# Autodesk Inventor assembly: Tracker
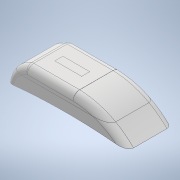
[picture p0: Inventor's stored thumbnail of the model, 180x180]
Saved by Autodesk Inventor 2020 (Build 240168000, 168)
## iProperties
Created: 2019-07-11
Part Number: Tracker
Document SubType Name: Assembly
Designer: tyrre
Author: tyrre
## Documents named in this file (6)
- C:\Users\tyrre\OneDrive\Desktop\University - Ryan\Work\Work - 2019\Inventor Files\Tracker V2\Tracker V2.iam
- C:\Users\tyrre\OneDrive\Desktop\University - Ryan\Work\Work - 2019\Inventor Files\Tracker V2\BatteryV2.ipt
- C:\Users\tyrre\OneDrive\Desktop\University - Ryan\Work\Work - 2019\Inventor Files\Tracker V2\GPSV2.ipt
- C:\Users\tyrre\OneDrive\Desktop\University - Ryan\Work\Work - 2019\Inventor Files\Tracker V2\MoteinoPCBV2.ipt
- C:\Users\tyrre\OneDrive\Desktop\University - Ryan\Work\Work - 2019\Inventor Files\Tracker V2\Case - BottomV2.ipt
- C:\Users\tyrre\OneDrive\Desktop\University - Ryan\Work\Work - 2019\Inventor Files\Tracker V2\Case - TopV2.ipt
## Components (5 placed, 5 different names)
1. Battery:1 — Mate:1, Flush:2, Flush:3, Flush:5, Mate:8, Mate:9
2. GPS:1 — Mate:2, Flush:4, Flush:5, Mate:6, Mate:7, Flush:6
3. MoteinoPCBV2:1 — Mate:1, Flush:2, Flush:3, Mate:2, Flush:4
4. Case - Top:1 — Mate:6, Mate:7, Mate:10, Flush:6
5. Case - Bottom:1 — Mate:8, Mate:9, Mate:10
## Relationships (12: Mate 7, Flush 5)
- Mate:1: Battery:1 ↔ MoteinoPCBV2:1
- Flush:2 (1.193 mm): Battery:1 ↔ MoteinoPCBV2:1
- Flush:3: Battery:1 ↔ MoteinoPCBV2:1
- Mate:2: GPS:1 ↔ MoteinoPCBV2:1
- Flush:4: GPS:1 ↔ MoteinoPCBV2:1
- Flush:5 (8.75 mm): Battery:1 ↔ GPS:1
- Mate:6: GPS:1 ↔ Case - Top:1
- Mate:7: GPS:1 ↔ Case - Top:1
- Mate:8: Battery:1 ↔ Case - Bottom:1
- Mate:9: Battery:1 ↔ Case - Bottom:1
- Mate:10: Case - Top:1 ↔ Case - Bottom:1
- Flush:6: GPS:1 ↔ Case - Top:1
